# Autodesk Inventor assembly: Assy_wrist_back
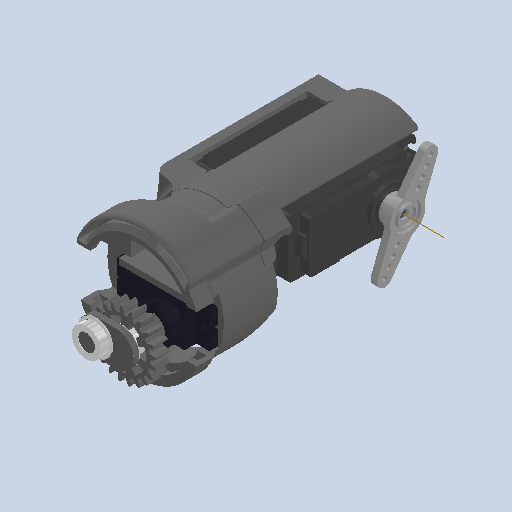
[picture p0: Inventor's stored thumbnail of the model, 512x512]
Saved by Autodesk Inventor 2024.1 (Build 281209000, 209)
## iProperties
Created: 2025-03-02
Part Number: Assy_wrist_back
Document SubType Name: Assembly
Designer: hibik
Author: hibik
## Documents named in this file (10)
- C:\Users\hibik\Documents\Robomech\RESCUE\ORCA\hard\arm\Assy_wrist_back.iam
- C:\Users\hibik\Documents\Robomech\RESCUE\ORCA\hard\std_parts\Miusei_ms18.ipt
- C:\Users\hibik\Documents\Robomech\RESCUE\ORCA\hard\arm\wrist_geard_hone.ipt
- C:\Users\hibik\Documents\Robomech\RESCUE\ORCA\hard\std_parts\bearing_6_10_3_MIR.ipt
- C:\Users\hibik\Documents\Robomech\RESCUE\ORCA\hard\arm\wrist_gear_spacer.ipt
- C:\Users\hibik\Documents\Robomech\RESCUE\ORCA\hard\arm\wrist_cover.ipt
- C:\Users\hibik\Documents\Robomech\RESCUE\ORCA\hard\std_parts\FS5103B.ipt
- C:\Users\hibik\Documents\Robomech\RESCUE\ORCA\hard\std_parts\feetech_servohone.ipt
- C:\Users\hibik\Documents\Robomech\RESCUE\ORCA\hard\arm\wrist_base.ipt
- C:\Users\hibik\Documents\Robomech\RESCUE\ORCA\hard\std_parts\bearing_6_10_3.ipt
## Components (10 placed, 9 different names)
1. wrist_base:1 — 挿入:9, メイト:1, メイト:2, メイト:3, メイト:4, フラッシュ:1, メイト:5, 挿入:15, 角度:3, フラッシュ:2
2. bearing_6_10_3:1 — 挿入:9
3. feetech_servohone:1 — 挿入:10, メイト:6
4. FS5103B:1 — 挿入:10, メイト:1, メイト:2, メイト:3
5. wrist_geard_hone:2 — 挿入:11, 挿入:14
6. wrist_gear_spacer:2 — 挿入:12, 挿入:13, 角度:2
7. bearing_6_10_3_MIR:3 — 挿入:13
8. bearing_6_10_3_MIR:4 — 挿入:11, 挿入:12
9. wrist_cover:2 — 挿入:15, 角度:1
10. Miusei_ms18:3 — 挿入:14, メイト:4, フラッシュ:1, メイト:5, 角度:1, 角度:2
## Relationships (18: Insert 7, Mate 6, Angle 3, Flush 2)
- 挿入:9 [Insert]: wrist_base:1 ↔ bearing_6_10_3:1
- 挿入:10 [Insert]: feetech_servohone:1 ↔ FS5103B:1
- メイト:1 [Mate]: wrist_base:1 ↔ FS5103B:1
- メイト:2 [Mate]: wrist_base:1 ↔ FS5103B:1
- メイト:3 [Mate]: wrist_base:1 ↔ FS5103B:1
- 挿入:11 [Insert]: wrist_geard_hone:2 ↔ bearing_6_10_3_MIR:4
- 挿入:12 [Insert]: wrist_gear_spacer:2 ↔ bearing_6_10_3_MIR:4
- 挿入:13 [Insert]: wrist_gear_spacer:2 ↔ bearing_6_10_3_MIR:3
- 挿入:14 [Insert]: wrist_geard_hone:2 ↔ Miusei_ms18:3
- メイト:4 [Mate]: wrist_base:1 ↔ Miusei_ms18:3
- フラッシュ:1 [Flush]: wrist_base:1 ↔ Miusei_ms18:3
- メイト:5 [Mate] (0.1 mm): wrist_base:1 ↔ Miusei_ms18:3
- 挿入:15 [Insert]: wrist_base:1 ↔ wrist_cover:2
- 角度:1 [Angle] (0 deg): wrist_cover:2 ↔ Miusei_ms18:3
- 角度:2 [Angle] (0 deg): wrist_gear_spacer:2 ↔ Miusei_ms18:3
- メイト:6 [Mate]: feetech_servohone:1
- 角度:3 [Angle] (0 deg): wrist_base:1
- フラッシュ:2 [Flush]: wrist_base:1
